# Autodesk Inventor assembly: Sensor_module_uCMotionBoard
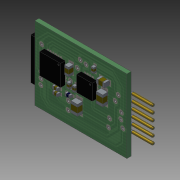
[picture p0: Inventor's stored thumbnail of the model, 180x180]
Saved by Autodesk Inventor 2013 (Build 170138000, 138)
## iProperties
Created: 2015-07-01
Part Number: Sensor_module_uCMotionBoard
Document SubType Name: Assembly
Designer: terg
Author: terg
## Documents named in this file (11)
- C:\Users\terg\Projects\ModularElectronics\3D_models\Sensor_module\Sensor_module_uCMotionBoard.iam
- C:\Users\terg\Projects\ModularElectronics\3D_models\Sensor_module\Sensor_module_uCMotionBoard_PCB.ipt
- C:\Users\terg\Projects\ModularElectronics\3D_models\Components\EFM32ZG110.ipt
- C:\Users\terg\Projects\ModularElectronics\3D_models\Components\0805_cap.ipt
- C:\Users\terg\Projects\ModularElectronics\3D_models\Components\0402_cap.ipt
- C:\Users\terg\Projects\ModularElectronics\3D_models\Components\0402_res.ipt
- C:\Users\terg\Projects\ModularElectronics\3D_models\Components\0603_cap.ipt
- C:\Users\terg\Projects\ModularElectronics\3D_models\Sensor_module\MPU6050.ipt
- C:\Users\terg\Projects\ModularElectronics\3D_models\Sensor_module\HMC5883L.ipt
- C:\Users\terg\Projects\ModularElectronics\3D_models\Components\FemalConnector.ipt
- C:\Users\terg\Projects\ModularElectronics\3D_models\Components\MaleConnector.ipt
## Components (23 placed, 10 different names)
1. Sensor_module_uCMotionBoard_PCB:1 — Zestawiający:1, Równoległy:1, Równoległy:2, Zestawiający:2, Zestawiający:3, Zestawiający:4, Zestawiający:5, Równoległy:3, Równoległy:4, Równoległy:5, Równoległy:6, Równoległy:7, Zestawiający:6, Zestawiający:7, Zestawiający:8, Zestawiający:9, Zestawiający:10, Równoległy:8, Równoległy:9, Równoległy:10, Równoległy:11, Równoległy:12, Równoległy:13, Równoległy:14, Zestawiający:11, Zestawiający:12, Zestawiający:13, Zestawiający:14, Zestawiający:15, Zestawiający:16, Zestawiający:17, Zestawiający:18, Zestawiający:19, Zestawiający:20, Równoległy:15, Równoległy:16, Równoległy:17, Równoległy:18, Zestawiający:21, Równoległy:19, Równoległy:20, Zestawiający:22, Równoległy:21, Równoległy:22, Zestawiający:23, Zestawiający:24
2. EFM32ZG110:1 — Zestawiający:1, Równoległy:1, Równoległy:2
3. 0805_cap:1 — Zestawiający:2, Równoległy:5, Równoległy:7
4. 0805_cap:2 — Zestawiający:3, Zestawiający:5, Równoległy:4
5. 0805_cap:3 — Zestawiający:4, Równoległy:3, Równoległy:6
6. 0402_cap:1 — Zestawiający:6, Równoległy:10, Równoległy:14
7. 0402_cap:2 — Zestawiający:7, Równoległy:11, Równoległy:13
8. 0402_cap:3 — Zestawiający:9, Równoległy:9, Równoległy:12
9. 0402_cap:4 — Zestawiający:8, Zestawiający:10, Równoległy:8
10. 0805_cap:4 — Zestawiający:12
11. 0805_cap:5 — Zestawiający:13
12. 0402_res:1 — Zestawiający:11
13. 0402_cap:5 — Zestawiający:14
14. 0402_cap:6 — Zestawiający:15
15. 0402_cap:7 — Zestawiający:16
16. 0402_cap:8 — Zestawiający:17
17. 0402_cap:9 — Zestawiający:18
18. 0603_cap:1 — Zestawiający:19, Równoległy:16, Równoległy:17
19. 0603_cap:2 — Zestawiający:20, Równoległy:15, Równoległy:18
20. MPU6050:1 — Zestawiający:21, Równoległy:19, Równoległy:20
21. HMC5883L:1 — Zestawiający:22, Równoległy:21, Równoległy:22
22. FemalConnector:1 — Zestawiający:23
23. MaleConnector:1 — Zestawiający:24
## Relationships (46: Mate 24, Flush 22)
- Zestawiający:1 [Mate]: Sensor_module_uCMotionBoard_PCB:1 ↔ EFM32ZG110:1
- Równoległy:1 [Flush] (5.515 mm): Sensor_module_uCMotionBoard_PCB:1 ↔ EFM32ZG110:1
- Równoległy:2 [Flush] (5.211 mm): Sensor_module_uCMotionBoard_PCB:1 ↔ EFM32ZG110:1
- Zestawiający:2 [Mate]: Sensor_module_uCMotionBoard_PCB:1 ↔ 0805_cap:1
- Zestawiający:3 [Mate]: Sensor_module_uCMotionBoard_PCB:1 ↔ 0805_cap:2
- Zestawiający:4 [Mate]: Sensor_module_uCMotionBoard_PCB:1 ↔ 0805_cap:3
- Zestawiający:5 [Mate] (-5.7 mm): Sensor_module_uCMotionBoard_PCB:1 ↔ 0805_cap:2
- Równoległy:3 [Flush] (1.238 mm): Sensor_module_uCMotionBoard_PCB:1 ↔ 0805_cap:3
- Równoległy:4 [Flush] (8.438 mm): Sensor_module_uCMotionBoard_PCB:1 ↔ 0805_cap:2
- Równoległy:5 [Flush] (11.455 mm): Sensor_module_uCMotionBoard_PCB:1 ↔ 0805_cap:1
- Równoległy:6 [Flush] (14.875 mm): Sensor_module_uCMotionBoard_PCB:1 ↔ 0805_cap:3
- Równoległy:7 [Flush] (6.634 mm): Sensor_module_uCMotionBoard_PCB:1 ↔ 0805_cap:1
- Zestawiający:6 [Mate]: Sensor_module_uCMotionBoard_PCB:1 ↔ 0402_cap:1
- Zestawiający:7 [Mate]: Sensor_module_uCMotionBoard_PCB:1 ↔ 0402_cap:2
- Zestawiający:8 [Mate]: Sensor_module_uCMotionBoard_PCB:1 ↔ 0402_cap:4
- Zestawiający:9 [Mate]: Sensor_module_uCMotionBoard_PCB:1 ↔ 0402_cap:3
- Zestawiający:10 [Mate] (-4.43 mm): Sensor_module_uCMotionBoard_PCB:1 ↔ 0402_cap:4
- Równoległy:8 [Flush] (7.023 mm): Sensor_module_uCMotionBoard_PCB:1 ↔ 0402_cap:4
- Równoległy:9 [Flush] (1.603 mm): Sensor_module_uCMotionBoard_PCB:1 ↔ 0402_cap:3
- Równoległy:10 [Flush] (9.136 mm): Sensor_module_uCMotionBoard_PCB:1 ↔ 0402_cap:1
- Równoległy:11 [Flush] (9.08 mm): Sensor_module_uCMotionBoard_PCB:1 ↔ 0402_cap:2
- Równoległy:12 [Flush] (9.754 mm): Sensor_module_uCMotionBoard_PCB:1 ↔ 0402_cap:3
- Równoległy:13 [Flush] (7.301 mm): Sensor_module_uCMotionBoard_PCB:1 ↔ 0402_cap:2
- Równoległy:14 [Flush] (9.253 mm): Sensor_module_uCMotionBoard_PCB:1 ↔ 0402_cap:1
- Zestawiający:11 [Mate]: Sensor_module_uCMotionBoard_PCB:1 ↔ 0402_res:1
- Zestawiający:12 [Mate]: Sensor_module_uCMotionBoard_PCB:1 ↔ 0805_cap:4
- Zestawiający:13 [Mate]: Sensor_module_uCMotionBoard_PCB:1 ↔ 0805_cap:5
- Zestawiający:14 [Mate]: Sensor_module_uCMotionBoard_PCB:1 ↔ 0402_cap:5
- Zestawiający:15 [Mate]: Sensor_module_uCMotionBoard_PCB:1 ↔ 0402_cap:6
- Zestawiający:16 [Mate]: Sensor_module_uCMotionBoard_PCB:1 ↔ 0402_cap:7
- Zestawiający:17 [Mate]: Sensor_module_uCMotionBoard_PCB:1 ↔ 0402_cap:8
- Zestawiający:18 [Mate]: Sensor_module_uCMotionBoard_PCB:1 ↔ 0402_cap:9
- Zestawiający:19 [Mate]: Sensor_module_uCMotionBoard_PCB:1 ↔ 0603_cap:1
- Zestawiający:20 [Mate]: Sensor_module_uCMotionBoard_PCB:1 ↔ 0603_cap:2
- Równoległy:15 [Flush] (2.759 mm): Sensor_module_uCMotionBoard_PCB:1 ↔ 0603_cap:2
- Równoległy:16 [Flush] (3.568 mm): Sensor_module_uCMotionBoard_PCB:1 ↔ 0603_cap:1
- Równoległy:17 [Flush] (6.564 mm): Sensor_module_uCMotionBoard_PCB:1 ↔ 0603_cap:1
- Równoległy:18 [Flush] (12.64 mm): Sensor_module_uCMotionBoard_PCB:1 ↔ 0603_cap:2
- Zestawiający:21 [Mate]: Sensor_module_uCMotionBoard_PCB:1 ↔ MPU6050:1
- Równoległy:19 [Flush] (1.829 mm): Sensor_module_uCMotionBoard_PCB:1 ↔ MPU6050:1
- Równoległy:20 [Flush] (3.713 mm): Sensor_module_uCMotionBoard_PCB:1 ↔ MPU6050:1
- Zestawiający:22 [Mate]: Sensor_module_uCMotionBoard_PCB:1 ↔ HMC5883L:1
- Równoległy:21 [Flush] (3.976 mm): Sensor_module_uCMotionBoard_PCB:1 ↔ HMC5883L:1
- Równoległy:22 [Flush] (8.861 mm): Sensor_module_uCMotionBoard_PCB:1 ↔ HMC5883L:1
- Zestawiający:23 [Mate]: Sensor_module_uCMotionBoard_PCB:1 ↔ FemalConnector:1
- Zestawiający:24 [Mate]: Sensor_module_uCMotionBoard_PCB:1 ↔ MaleConnector:1
